# Autodesk Inventor assembly: s-assy-gripper
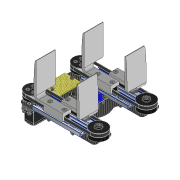
[picture p0: Inventor's stored thumbnail of the model, 180x180]
Saved by Autodesk Inventor 2022 (Build 260153000, 153)
## iProperties
Created: 2021-08-06
Part Number: s-assy-gripper
Document SubType Name: Assembly
Designer: yuta0
Mass: 593.374 g
Surface Area: 2184.28 cm^2
Volume: 287.927 cm^3
Density: 2.06085 g/cm^3
Author: yuta0
## Documents named in this file (22)
- C:\Users\yuta0\Documents\GitHub\catchrobo_hardware\assy-scara\s-assy-gripper.iam
- C:\Users\yuta0\Documents\GitHub\catchrobo_hardware\assy-scara\carbon_plate14.ipt
- C:\Users\yuta0\Documents\GitHub\catchrobo_hardware\assy-scara\mrs20-100.ipt
- C:\Users\yuta0\Documents\GitHub\catchrobo_hardware\assy-scara\mr-20cs_1.iam
- C:\Users\yuta0\Documents\GitHub\catchrobo_hardware\assy-scara\belt4.ipt
- C:\Users\yuta0\Documents\GitHub\catchrobo_hardware\assy-scara\base37.ipt
- C:\Users\yuta0\Documents\GitHub\catchrobo_hardware\assy-scara\USB Cam model ELP-USBFHD01M-L21.ipt
- C:\Users\yuta0\Documents\GitHub\catchrobo_hardware\assy-scara\CB3-5.ipt
- C:\Users\yuta0\Documents\GitHub\catchrobo_hardware\assy-scara\LBNR4.ipt
- C:\Users\yuta0\Documents\GitHub\catchrobo_hardware\assy-scara\ARU-2010.ipt
- C:\Users\yuta0\Documents\GitHub\catchrobo_hardware\assy-scara\CB2-4.ipt
- C:\Users\yuta0\Documents\GitHub\catchrobo_hardware\assy-scara\d_type_board.ipt
- C:\Users\yuta0\Documents\GitHub\catchrobo_hardware\assy-scara\hexagonal_spacer_M3_5mm.ipt
- C:\Users\yuta0\Documents\GitHub\catchrobo_hardware\assy-scara\LBNR3.ipt
- C:\Users\yuta0\Documents\GitHub\catchrobo_hardware\assy-scara\s-assy-rc_servo.iam
- C:\Users\yuta0\Documents\GitHub\catchrobo_hardware\assy-scara\s-assy-gripper_tentioner.iam
- C:\Users\yuta0\Documents\GitHub\catchrobo_hardware\assy-scara\FU650AD5-C6.ipt
- C:\Users\yuta0\Documents\GitHub\catchrobo_hardware\assy-scara\base21.ipt
- C:\Users\yuta0\Documents\GitHub\catchrobo_hardware\assy-scara\CBSTSR4-14.ipt
- C:\Users\yuta0\Documents\GitHub\catchrobo_hardware\assy-scara\base49.ipt
- C:\Users\yuta0\Documents\GitHub\catchrobo_hardware\assy-scara\scara-base26.ipt
- C:\Users\yuta0\Documents\GitHub\catchrobo_hardware\assy-scara\CBSTSR4-20.ipt
## Components (72 placed, 21 different names)
1. carbon_plate14:1 — メイト:1, メイト:2, メイト:3, メイト:51, メイト:52, メイト:53, メイト:90, メイト:92, 角度:1, メイト:98, メイト:102, メイト:103, メイト:104, メイト:105, メイト:106, メイト:107, メイト:109, メイト:110, メイト:111, メイト:113, メイト:139, メイト:140, メイト:141, メイト:142, メイト:143, メイト:144, メイト:147, メイト:150, メイト:183, メイト:197, メイト:200, 角度:4, 角度:5, メイト:201, メイト:202, メイト:203, メイト:207, メイト:208
2. s-assy-rc_servo:1 [sub-assembly] — メイト:139, メイト:140, メイト:141, メイト:145, メイト:146, メイト:247
3. s-assy-rc_servo:2 [sub-assembly] — メイト:142, メイト:143, メイト:144, メイト:153, メイト:154, メイト:248, メイト:249
4. s-assy-gripper_tentioner:1 [sub-assembly] — メイト:147, メイト:149
5. USB Cam model ELP-USBFHD01M-L21:1 — メイト:51, メイト:52, メイト:53, メイト:99, メイト:100, メイト:101
6. hexagonal_spacer_M3_5mm:1 — メイト:106, メイト:107, メイト:108, メイト:114
7. LBNR3:1 — メイト:108, メイト:109
8. LBNR3:2 — メイト:112, メイト:113
9. hexagonal_spacer_M3_5mm:2 — メイト:110, メイト:111, メイト:112
10. d_type_board:1 — メイト:104, メイト:105, メイト:114, メイト:115, メイト:116, メイト:117, メイト:118
11. CB3-5:11 — メイト:115, メイト:116
12. CB3-5:12 — メイト:117, メイト:118
13. belt4:1 — メイト:145, メイト:146, メイト:149
14. belt4:2 — メイト:152, メイト:153, メイト:154, メイト:234
15. FU650AD5-C6:1 — メイト:197, メイト:198, 角度:5
16. FU650AD5-C6:2 — メイト:199, メイト:200, 角度:4
17. base21:1 — メイト:201, メイト:202, メイト:203, メイト:204, メイト:205
18. base21:2 — メイト:206, メイト:207, メイト:208, メイト:209, メイト:210
19. scara-base26:1 — メイト:247, メイト:248, メイト:249
20. s-assy-gripper_tentioner:2 [sub-assembly] — メイト:150, メイト:152
21. ARU-2010:1 — メイト:98, メイト:99
22. CB2-4:1 — メイト:100, メイト:101
23. CB2-4:2 — メイト:102, メイト:103
24. ARU-2010:2
25. CB2-4:3
26. CB2-4:6
27. ARU-2010:3
28. CB2-4:4
29. CB2-4:7
30. ARU-2010:4
31. CB2-4:5
32. CB2-4:8
33. base49:1 — メイト:227, メイト:234, 正接:1, メイト:251, メイト:253
34. CBSTSR4-20:2 — メイト:252, メイト:253
35. CBSTSR4-20:1 — メイト:250, メイト:251
36. mr-20cs_1:2 [sub-assembly] — メイト:226
37. mrs20-100:2 — メイト:183, メイト:198
38. CBSTSR4-14:2
39. LBNR4:3 — メイト:205
40. CBSTSR4-14:1
41. LBNR4:4 — メイト:204
42. base37:2 — メイト:226, メイト:227, 正接:1, メイト:250, メイト:252
43. base49:4 — フラッシュ:6
44. CBSTSR4-20:5
45. CBSTSR4-20:6
46. mr-20cs_1:3 [sub-assembly]
47. mrs20-100:3
48. CBSTSR4-14:5
49. LBNR4:5
50. CBSTSR4-14:6
51. LBNR4:6
52. base37:4
53. base49:3 — フラッシュ:4, メイト:242, メイト:255, メイト:257, フラッシュ:5, フラッシュ:6
54. CBSTSR4-20:3 — メイト:254, メイト:255
55. CBSTSR4-20:4 — メイト:256, メイト:257
56. mr-20cs_1:1 [sub-assembly] — メイト:7, メイト:8, メイト:45, メイト:46, メイト:47
57. mrs20-100:1 — メイト:1, メイト:2, メイト:3, メイト:7, メイト:8, メイト:199
58. LBNR4:1 — メイト:90, 角度:2, メイト:210
59. CBSTSR4-14:3
60. CBSTSR4-14:4 — メイト:206
61. LBNR4:2 — メイト:92, 角度:1, 角度:2, メイト:209
62. base37:1 — メイト:45, メイト:46, メイト:47, フラッシュ:4, メイト:242, メイト:254, メイト:256, フラッシュ:5
63. base49:5
64. CBSTSR4-20:7
65. CBSTSR4-20:8
66. mr-20cs_1:4 [sub-assembly]
67. mrs20-100:4
68. LBNR4:7
69. CBSTSR4-14:7
70. CBSTSR4-14:8
71. LBNR4:8
72. base37:3
## Component patterns: (4 elements, first: ARU-2010:1 + CB2-4:1 + CB2-4:2), (2 elements, first: base49:1 + CBSTSR4-20:2 + CBSTSR4-20:1 + mr-20cs_1:2 + mrs20-100:2 + CBSTSR4-14:2 + LBNR4:3 + CBSTSR4-14:1 + LBNR4:4 + base37:2), (2 elements, first: base49:3 + CBSTSR4-20:3 + CBSTSR4-20:4 + mr-20cs_1:1 + mrs20-100:1 + LBNR4:1 + CBSTSR4-14:3 + CBSTSR4-14:4 + LBNR4:2 + base37:1)
## Relationships (103: Mate 93, Angle 5, Flush 4, Tangent 1)
- [Flush] (-17.5 mm): mr-20cs_1:2 ↔ mrs20-100:2
- メイト:1 [Mate]: carbon_plate14:1 ↔ mrs20-100:1
- メイト:2 [Mate]: carbon_plate14:1 ↔ mrs20-100:1
- メイト:3 [Mate]: carbon_plate14:1 ↔ mrs20-100:1
- メイト:7 [Mate] (0.1 mm): mr-20cs_1:1 ↔ mrs20-100:1
- メイト:8 [Mate] (0.15 mm): mr-20cs_1:1 ↔ mrs20-100:1
- メイト:45 [Mate]: mr-20cs_1:1 ↔ base37:1
- メイト:46 [Mate]: mr-20cs_1:1 ↔ base37:1
- メイト:47 [Mate]: mr-20cs_1:1 ↔ base37:1
- メイト:51 [Mate] (10 mm): carbon_plate14:1 ↔ USB Cam model ELP-USBFHD01M-L21:1
- メイト:52 [Mate]: carbon_plate14:1 ↔ USB Cam model ELP-USBFHD01M-L21:1
- メイト:53 [Mate]: carbon_plate14:1 ↔ USB Cam model ELP-USBFHD01M-L21:1
- メイト:90 [Mate]: carbon_plate14:1 ↔ LBNR4:1
- メイト:92 [Mate]: carbon_plate14:1 ↔ LBNR4:2
- 角度:1 [Angle] (0 deg): carbon_plate14:1 ↔ LBNR4:2
- 角度:2 [Angle] (0 deg): LBNR4:1 ↔ LBNR4:2
- メイト:98 [Mate]: carbon_plate14:1 ↔ ARU-2010:1
- メイト:99 [Mate]: USB Cam model ELP-USBFHD01M-L21:1 ↔ ARU-2010:1
- メイト:100 [Mate]: USB Cam model ELP-USBFHD01M-L21:1 ↔ CB2-4:1
- メイト:101 [Mate]: USB Cam model ELP-USBFHD01M-L21:1 ↔ CB2-4:1
- メイト:102 [Mate]: carbon_plate14:1 ↔ CB2-4:2
- メイト:103 [Mate]: carbon_plate14:1 ↔ CB2-4:2
- メイト:104 [Mate]: carbon_plate14:1 ↔ d_type_board:1
- メイト:105 [Mate]: carbon_plate14:1 ↔ d_type_board:1
- メイト:106 [Mate]: carbon_plate14:1 ↔ hexagonal_spacer_M3_5mm:1
- メイト:107 [Mate]: carbon_plate14:1 ↔ hexagonal_spacer_M3_5mm:1
- メイト:108 [Mate]: hexagonal_spacer_M3_5mm:1 ↔ LBNR3:1
- メイト:109 [Mate]: carbon_plate14:1 ↔ LBNR3:1
- メイト:110 [Mate]: carbon_plate14:1 ↔ hexagonal_spacer_M3_5mm:2
- メイト:111 [Mate]: carbon_plate14:1 ↔ hexagonal_spacer_M3_5mm:2
- メイト:112 [Mate]: LBNR3:2 ↔ hexagonal_spacer_M3_5mm:2
- メイト:113 [Mate]: carbon_plate14:1 ↔ LBNR3:2
- メイト:114 [Mate]: hexagonal_spacer_M3_5mm:1 ↔ d_type_board:1
- メイト:115 [Mate]: d_type_board:1 ↔ CB3-5:11
- メイト:116 [Mate]: d_type_board:1 ↔ CB3-5:11
- メイト:117 [Mate]: d_type_board:1 ↔ CB3-5:12
- メイト:118 [Mate]: d_type_board:1 ↔ CB3-5:12
- [Mate]: mrs20-100:1 ↔ CBSTSR4-14:3
- [Mate]: mrs20-100:1 ↔ CBSTSR4-14:3
- [Mate]: mrs20-100:1 ↔ CBSTSR4-14:4
- [Mate]: mrs20-100:1 ↔ CBSTSR4-14:4
- メイト:139 [Mate]: carbon_plate14:1 ↔ s-assy-rc_servo:1
- メイト:140 [Mate]: carbon_plate14:1 ↔ s-assy-rc_servo:1
- メイト:141 [Mate]: carbon_plate14:1 ↔ s-assy-rc_servo:1
- メイト:142 [Mate]: carbon_plate14:1 ↔ s-assy-rc_servo:2
- メイト:143 [Mate]: carbon_plate14:1 ↔ s-assy-rc_servo:2
- メイト:144 [Mate]: carbon_plate14:1 ↔ s-assy-rc_servo:2
- メイト:145 [Mate]: s-assy-rc_servo:1 ↔ belt4:1
- メイト:146 [Mate] (0.5 mm): s-assy-rc_servo:1 ↔ belt4:1
- メイト:147 [Mate]: carbon_plate14:1 ↔ s-assy-gripper_tentioner:1
- メイト:149 [Mate]: s-assy-gripper_tentioner:1 ↔ belt4:1
- メイト:150 [Mate]: carbon_plate14:1 ↔ s-assy-gripper_tentioner:2
- メイト:152 [Mate]: belt4:2 ↔ s-assy-gripper_tentioner:2
- メイト:153 [Mate]: s-assy-rc_servo:2 ↔ belt4:2
- メイト:154 [Mate] (0.5 mm): s-assy-rc_servo:2 ↔ belt4:2
- [Mate] (0.1 mm): mr-20cs_1:2 ↔ mrs20-100:2
- [Mate] (0.15 mm): mr-20cs_1:2 ↔ mrs20-100:2
- [Mate]: mr-20cs_1:2 ↔ base37:2
- [Angle] (0 deg): LBNR4:3 ↔ LBNR4:4
- [Mate]: mrs20-100:2 ↔ CBSTSR4-14:2
- [Mate]: mrs20-100:2 ↔ CBSTSR4-14:2
- [Mate]: mrs20-100:2 ↔ CBSTSR4-14:1
- [Mate]: mrs20-100:2 ↔ CBSTSR4-14:1
- [Mate]: carbon_plate14:1 ↔ CBSTSR4-14:2
- [Mate]: carbon_plate14:1 ↔ CBSTSR4-14:1
- メイト:183 [Mate]: carbon_plate14:1 ↔ mrs20-100:2
- [Mate]: CBSTSR4-14:1 ↔ LBNR4:4
- [Mate]: CBSTSR4-14:2 ↔ LBNR4:3
- メイト:197 [Mate]: carbon_plate14:1 ↔ FU650AD5-C6:1
- メイト:198 [Mate]: FU650AD5-C6:1 ↔ mrs20-100:2
- メイト:199 [Mate]: FU650AD5-C6:2 ↔ mrs20-100:1
- メイト:200 [Mate]: carbon_plate14:1 ↔ FU650AD5-C6:2
- 角度:4 [Angle] (0 deg): carbon_plate14:1 ↔ FU650AD5-C6:2
- 角度:5 [Angle] (0 deg): carbon_plate14:1 ↔ FU650AD5-C6:1
- メイト:201 [Mate]: carbon_plate14:1 ↔ base21:1
- メイト:202 [Mate]: carbon_plate14:1 ↔ base21:1
- メイト:203 [Mate]: carbon_plate14:1 ↔ base21:1
- メイト:204 [Mate]: base21:1 ↔ LBNR4:4
- メイト:205 [Mate]: base21:1 ↔ LBNR4:3
- メイト:206 [Mate]: base21:2 ↔ CBSTSR4-14:4
- メイト:207 [Mate]: carbon_plate14:1 ↔ base21:2
- メイト:208 [Mate]: carbon_plate14:1 ↔ base21:2
- メイト:209 [Mate]: base21:2 ↔ LBNR4:2
- メイト:210 [Mate]: base21:2 ↔ LBNR4:1
- メイト:226 [Mate]: mr-20cs_1:2 ↔ base37:2
- メイト:227 [Mate]: base49:1 ↔ base37:2
- メイト:234 [Mate]: belt4:2 ↔ base49:1
- 正接:1 [Tangent]: base49:1 ↔ base37:2
- フラッシュ:4 [Flush] (-3 mm): base49:3 ↔ base37:1
- メイト:242 [Mate]: base49:3 ↔ base37:1
- メイト:247 [Mate]: s-assy-rc_servo:1 ↔ scara-base26:1
- メイト:248 [Mate]: s-assy-rc_servo:2 ↔ scara-base26:1
- メイト:249 [Mate]: s-assy-rc_servo:2 ↔ scara-base26:1
- メイト:250 [Mate]: CBSTSR4-20:1 ↔ base37:2
- メイト:251 [Mate]: base49:1 ↔ CBSTSR4-20:1
- メイト:252 [Mate]: CBSTSR4-20:2 ↔ base37:2
- メイト:253 [Mate]: base49:1 ↔ CBSTSR4-20:2
- メイト:254 [Mate]: CBSTSR4-20:3 ↔ base37:1
- メイト:255 [Mate]: base49:3 ↔ CBSTSR4-20:3
- メイト:256 [Mate]: CBSTSR4-20:4 ↔ base37:1
- メイト:257 [Mate]: base49:3 ↔ CBSTSR4-20:4
- フラッシュ:5 [Flush]: base49:3 ↔ base37:1
- フラッシュ:6 [Flush]: base49:4 ↔ base49:3
## Named parameters: d280_d22 = 0.1 mm, d281_d23 = 0.15 mm, d282_d214 = 0 mm, d283_d215 = 0 mm, d284_d216 = 0 mm, d285_d217 = 0 mm, d286_d170 = 0 deg, d289_d106 = 0 mm, d297_d26 = -17.5 mm
